# Autodesk Inventor assembly: Pressure sensor
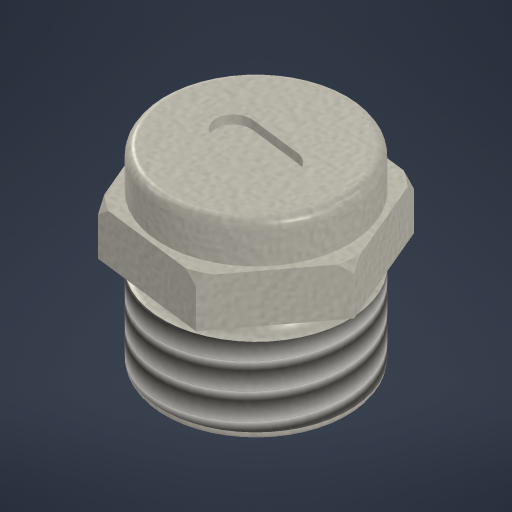
[picture p0: Inventor's stored thumbnail of the model, 512x512]
Saved by Autodesk Inventor 2023 (Build 270158000, 158)
## iProperties
Created: 2022-08-25
Part Number: Pressure sensor
Document SubType Name: Assembly
Designer: Mike
Author: Mike
## Documents named in this file (3)
- C:\Users\Mike\Desktop\Mechatronics\Mechatronics 5.1\Liquid-engine-cooling-system\design files\Ethanol engine 5 -inventor\Pressure sensor.iam
- C:\Users\Mike\Desktop\Mechatronics\Mechatronics 5.1\Liquid-engine-cooling-system\design files\Ethanol engine 5 -inventor\Pressure sensor.ipt
- C:\Users\Mike\Desktop\Mechatronics\Mechatronics 5.1\Liquid-engine-cooling-system\design files\Ethanol engine 5 -inventor\Pressure sensor connector.ipt
## Components (2 placed, 2 different names)
1. Pressure sensor:1 — Mate:1, Mate:2, Mate:3
2. Pressure sensor connector:1 — Mate:1, Mate:2, Mate:3
## Relationships (3: Mate 3)
- Mate:1: Pressure sensor:1 ↔ Pressure sensor connector:1
- Mate:2: Pressure sensor:1 ↔ Pressure sensor connector:1
- Mate:3: Pressure sensor:1 ↔ Pressure sensor connector:1
